# Autodesk Inventor assembly: 090 ASY bottom
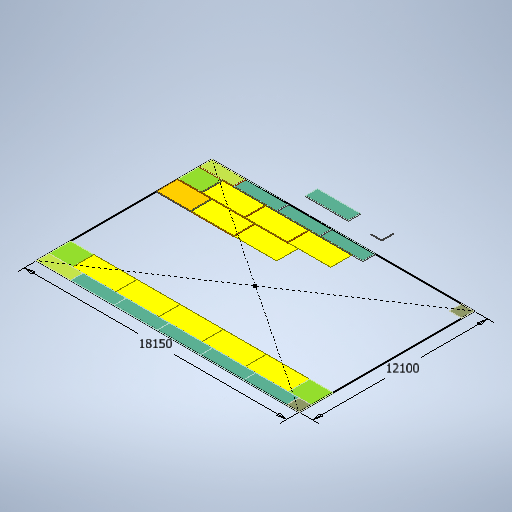
[picture p0: Inventor's stored thumbnail of the model, 512x512]
Saved by Autodesk Inventor 2026.2 (Build 302298000, 298)
## iProperties
Created: 2026-05-19
Part Number: 090 ASY bottom
Document SubType Name: Assembly
Designer: user
Author: user
## Documents named in this file (15)
- C:\Users\admin\Documents\Inventor\GBK-Gubkinskiy\090 ASY bottom.iam
- C:\Users\admin\Documents\Inventor\GBK-Gubkinskiy\Пол\0921_CPY1.ipt
- C:\Users\admin\Documents\Inventor\GBK-Gubkinskiy\Пол\0923_CPY1.ipt
- C:\Users\admin\Documents\Inventor\GBK-Gubkinskiy\Пол\GBK bottom 0124.ipt
- C:\Users\admin\Documents\Inventor\GBK-Gubkinskiy\Пол\GBK bottom 0113.ipt
- C:\Users\admin\Documents\Inventor\GBK-Gubkinskiy\Пол\GBK bottom 0131.ipt
- C:\Users\admin\Documents\Inventor\GBK-Gubkinskiy\Пол\0921_CPY.ipt
- C:\Users\admin\Documents\Inventor\GBK-Gubkinskiy\Пол\0923_CPY.ipt
- C:\Users\admin\Documents\Inventor\GBK-Gubkinskiy\Пол\0921_CPY1_CPY.ipt
- C:\Users\admin\Documents\Inventor\GBK-Gubkinskiy\Пол\GBK bottom 0231.ipt
- C:\Users\admin\Documents\Inventor\GBK-Gubkinskiy\Пол\GBK bottom 0127.ipt
- C:\Users\admin\Documents\Inventor\GBK-Gubkinskiy\ASY GBK bottom 0010.iam
- C:\Users\admin\Documents\Inventor\GBK-Gubkinskiy\Пол\GBK bottom 0133.ipt
- C:\Users\admin\Documents\Inventor\GBK-Gubkinskiy\ASY GBK bottom 0020.iam
- C:\Users\admin\Documents\Inventor\GBK-Gubkinskiy\Пол\GBK bottom 0128.ipt
## Components (43 placed, 14 different names)
1. 0923_CPY:1 — Rigid:43, Mate:13, Mate:14
2. GBK bottom 0131:1 — Rigid:43, Mate:15
3. GBK bottom 0113:1 — Rigid:21
4. 0921_CPY1:1 — Rigid:13, Mate:2, Mate:3, Mate:13, Mate:14, Mate:15
5. GBK bottom 0123:5 — Rigid:21
6. GBK bottom 0124:3 — Rigid:36
7. 0921_CPY:11
8. 0921_CPY:12
9. 0921_CPY:13
10. 0921_CPY:14
11. 0921_CPY:15
12. GBK bottom 0124:4
13. 0921_CPY1:2 — Rigid:36
14. GBK bottom 0113:2
15. GBK bottom 0123:6
16. GBK bottom 0123:7
17. GBK bottom 0123:8
18. GBK bottom 0123:9
19. GBK bottom 0123:10
20. 0923_CPY1:1 — Mate:5, Rigid:41
21. GBK bottom 0231:1 — Rigid:15, Rigid:39, Mate:10, Mate:11, Mate:12
22. GBK bottom 0127:1 — Rigid:22
23. GBK bottom 0124:2 — Rigid:7
24. 0921_CPY:10 — Rigid:22
25. 0921_CPY:5 — Rigid:6, Rigid:7
26. 0921_CPY:9
27. 0921_CPY:4 — Rigid:5, Rigid:6
28. 0921_CPY:8
29. 0921_CPY:3 — Rigid:5, Rigid:38
30. 0921_CPY:7 — Rigid:40
31. ASY GBK bottom 0010:3 [sub-assembly] — Rigid:39, Rigid:40
32. ASY GBK bottom 0010:2 [sub-assembly] — Rigid:37, Rigid:38
33. GBK bottom 0131:2 — Rigid:44, Mate:12
34. 0923_CPY1:2 — Rigid:44, Mate:10, Mate:11
35. GBK 0214  bottom:1 — Mate:4, Rigid:41, Mate:6
36. ASY GBK bottom 0010:1 [sub-assembly] — Rigid:37
37. GBK bottom 0124:1 — Mate:1, Rigid:13, Rigid:15, Mate:4, Mate:5, Mate:6
38. ASY GBK bottom 0020:1 [sub-assembly] — Rigid:45
39. ASY GBK bottom 0020:2 [sub-assembly] — Rigid:45, Rigid:46
40. ASY GBK bottom 0020:3 [sub-assembly] — Rigid:46
41. ASY GBK bottom 0020:4 [sub-assembly]
42. GBK bottom 0128:1 — Rigid:47
43. 0923_CPY:2 — Rigid:47
## Relationships (47: WeldJoint 35, Mate 12)
- [WeldJoint] (4 mm): ASY GBK bottom 0010:1 ↔ GBK bottom 0124:1
- Rigid:5 [WeldJoint] (4 mm): 0921_CPY:4 ↔ 0921_CPY:3
- Rigid:6 [WeldJoint] (4 mm): 0921_CPY:5 ↔ 0921_CPY:4
- Rigid:7 [WeldJoint] (4 mm): GBK bottom 0124:2 ↔ 0921_CPY:5
- Mate:1 (-9075 mm): GBK bottom 0124:1
- [WeldJoint] (4 mm): 0921_CPY:8 ↔ 0921_CPY:7
- [WeldJoint] (4 mm): 0921_CPY:9 ↔ 0921_CPY:8
- [WeldJoint] (4 mm): 0921_CPY:10 ↔ 0921_CPY:9
- Rigid:13 [WeldJoint] (4 mm): 0921_CPY1:1 ↔ GBK bottom 0124:1
- Mate:2: 0921_CPY1:1
- Mate:3 (-6050 mm): 0921_CPY1:1
- [WeldJoint] (4 mm): 0921_CPY1:1 ↔ ASY GBK bottom 0020:1
- Rigid:15 [WeldJoint] (4 mm): GBK bottom 0231:1 ↔ GBK bottom 0124:1
- Rigid:21 [WeldJoint] (4 mm): GBK bottom 0113:1 ↔ GBK bottom 0123:5
- Rigid:22 [WeldJoint] (4 mm): GBK bottom 0127:1 ↔ 0921_CPY:10
- [WeldJoint] (4 mm): GBK bottom 0124:3 ↔ 0921_CPY:11
- [WeldJoint] (4 mm): 0921_CPY:11 ↔ 0921_CPY:12
- [WeldJoint] (4 mm): 0921_CPY:12 ↔ 0921_CPY:13
- [WeldJoint] (4 mm): 0921_CPY:13 ↔ 0921_CPY:14
- [WeldJoint] (4 mm): 0921_CPY:14 ↔ 0921_CPY:15
- [WeldJoint] (4 mm): 0921_CPY:15 ↔ GBK bottom 0124:4
- [WeldJoint] (4 mm): 0921_CPY1:2 ↔ GBK bottom 0123:6
- [WeldJoint] (4 mm): GBK bottom 0123:6 ↔ GBK bottom 0123:7
- [WeldJoint] (4 mm): GBK bottom 0123:7 ↔ GBK bottom 0123:8
- [WeldJoint] (4 mm): GBK bottom 0123:8 ↔ GBK bottom 0123:9
- [WeldJoint] (4 mm): GBK bottom 0123:9 ↔ GBK bottom 0123:10
- [WeldJoint] (4 mm): GBK bottom 0113:2 ↔ GBK bottom 0123:10
- Rigid:36 [WeldJoint] (4 mm): GBK bottom 0124:3 ↔ 0921_CPY1:2
- Rigid:37 [WeldJoint] (4 mm): ASY GBK bottom 0010:2 ↔ ASY GBK bottom 0010:1
- Rigid:38 [WeldJoint] (4 mm): 0921_CPY:3 ↔ ASY GBK bottom 0010:2
- Rigid:39 [WeldJoint] (4 mm): GBK bottom 0231:1 ↔ ASY GBK bottom 0010:3
- Rigid:40 [WeldJoint] (4 mm): 0921_CPY:7 ↔ ASY GBK bottom 0010:3
- Mate:4: GBK 0214  bottom:1 ↔ GBK bottom 0124:1
- Mate:5 (-30 mm): 0923_CPY1:1 ↔ GBK bottom 0124:1
- Rigid:41 [WeldJoint]: 0923_CPY1:1 ↔ GBK 0214  bottom:1
- Mate:6 (-30 mm): GBK 0214  bottom:1 ↔ GBK bottom 0124:1
- Rigid:43 [WeldJoint]: 0923_CPY:1 ↔ GBK bottom 0131:1
- Rigid:44 [WeldJoint]: GBK bottom 0131:2 ↔ 0923_CPY1:2
- Mate:10: GBK bottom 0231:1 ↔ 0923_CPY1:2
- Mate:11 (-30 mm): GBK bottom 0231:1 ↔ 0923_CPY1:2
- Mate:12 (-30 mm): GBK bottom 0231:1 ↔ GBK bottom 0131:2
- Mate:13: 0923_CPY:1 ↔ 0921_CPY1:1
- Mate:14 (-30 mm): 0923_CPY:1 ↔ 0921_CPY1:1
- Mate:15 (-30 mm): GBK bottom 0131:1 ↔ 0921_CPY1:1
- Rigid:45 [WeldJoint] (4 mm): ASY GBK bottom 0020:1 ↔ ASY GBK bottom 0020:2
- Rigid:46 [WeldJoint] (4 mm): ASY GBK bottom 0020:2 ↔ ASY GBK bottom 0020:3
- Rigid:47 [WeldJoint]: GBK bottom 0128:1 ↔ 0923_CPY:2
## Named parameters: d65_d59 = 4 mm, d66_d60 = 4 mm, d67_d61 = 4 mm, d85_d37 = 4 mm, d86_d58 = 4 mm, d87_d59 = 4 mm, d88_d60 = 4 mm, d89_d61 = 4 mm, d90_d62 = 4 mm, d96_d76 = 4 mm, d97_d79 = 4 mm, d98_d80 = 4 mm, d99_d81 = 4 mm, d100_d82 = 4 mm, d101_d83 = 4 mm
